# Autodesk Inventor assembly: 1Sborka antenn
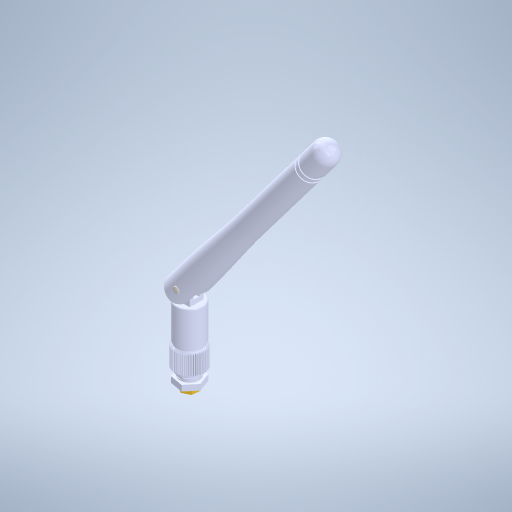
[picture p0: Inventor's stored thumbnail of the model, 512x512]
Saved by Autodesk Inventor 2024 (Build 280153000, 153)
## iProperties
Created: 2023-11-30
Part Number: 1Sborka antenn
Description: STEP AP214
Document SubType Name: Assembly
Designer: Roman Suk
Sending System: SolidWorks 2020
Preprocessor: SwSTEP 2.0
Title: 1Sborka antenn.STEP
Author: admin
Revision Number: ANY
## Documents named in this file (6)
- C:\Users\Roman Suk\Documents\Ročníkovka SŠ\Technical documentation\Final\1assemble antenn\1assemble antenn.iam
- C:\Users\Roman Suk\Documents\Ročníkovka SŠ\Technical documentation\Final\1assemble antenn\antenn2.ipt
- C:\Users\Roman Suk\Documents\Ročníkovka SŠ\Technical documentation\Final\1assemble antenn\antenn1.ipt
- C:\Users\Roman Suk\Documents\Ročníkovka SŠ\Technical documentation\Final\1assemble antenn\part3.ipt
- C:\Users\Roman Suk\Documents\Ročníkovka SŠ\Technical documentation\Final\1assemble antenn\part4.ipt
- C:\Users\Roman Suk\Documents\Ročníkovka SŠ\Technical documentation\Final\1assemble antenn\taper pin unhardened_iso_ISO 2339 - A - 2 x 10 - St.ipt
## Components (5 placed, 5 different names)
1. antenn2_1 — Insert:1, Insert:2, Insert:3
2. antenn1_2 — Insert:2
3. part3_3 — Mate:1, Mate:2
4. part4_4 — Mate:1, Insert:3, Mate:2
5. taper pin unhardened_iso_ISO 2339 - A - 2 x 10 - St_5 — Insert:1
## Relationships (5: Insert 3, Mate 2)
- Insert:1 (-2.5 mm): antenn2_1 ↔ taper pin unhardened_iso_ISO 2339 - A - 2 x 10 - St_5
- Insert:2: antenn2_1 ↔ antenn1_2
- Mate:1: part3_3 ↔ part4_4
- Insert:3: antenn2_1 ↔ part4_4
- Mate:2: part3_3 ↔ part4_4
